# Autodesk Inventor assembly: 520 DC Gear Motor Bracket Assembly
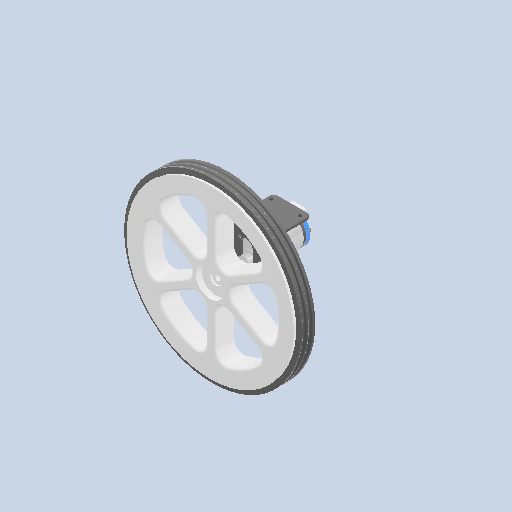
[picture p0: Inventor's stored thumbnail of the model, 512x512]
Saved by Autodesk Inventor 2025.2 (Build 292293000, 293)
## iProperties
Created: 2025-01-16
Part Number: 520 DC Gear Motor Bracket Assembly
Document SubType Name: Assembly
Designer: Matt Tidd
Author: Matt Tidd
## Documents named in this file (6)
- C:\mnguyen\H2A\cad\Motors_and_Wheels\Wheel Assembly\Motor Wheel Assembly.iam
- C:\mnguyen\H2A\cad\Motors_and_Wheels\520 DC Gear Motor Bracket.ipt
- C:\mnguyen\H2A\cad\Motors_and_Wheels\520 DC Gear Motor.ipt
- C:\mnguyen\H2A\cad\Motors_and_Wheels\Wheel Assembly\520 DC Gear Motor Wheel Coupler.ipt
- C:\mnguyen\H2A\cad\Motors_and_Wheels\Wheel Assembly\PLA Wheel Frame.ipt
- C:\mnguyen\H2A\cad\Motors_and_Wheels\Wheel Assembly\TPU Tire.ipt
## Components (5 placed, 5 different names)
1. 520 DC Gear Motor Wheel Coupler:1 — Rotational:2, Rigid:1
2. PLA Wheel Frame:1 — Rigid:1, Rigid:2
3. TPU Tire:1 — Rigid:2
4. 520 DC Gear Motor Bracket:1 — Rotational:1
5. 520 DC Gear Motor:1 — Rotational:1, Rotational:2
## Relationships (4: RevoluteJoint 2, WeldJoint 2)
- Rotational:1 [RevoluteJoint]: 520 DC Gear Motor Bracket:1 ↔ 520 DC Gear Motor:1
- Rotational:2 [RevoluteJoint]: 520 DC Gear Motor Wheel Coupler:1 ↔ 520 DC Gear Motor:1
- Rigid:1 [WeldJoint]: 520 DC Gear Motor Wheel Coupler:1 ↔ PLA Wheel Frame:1
- Rigid:2 [WeldJoint]: PLA Wheel Frame:1 ↔ TPU Tire:1
